# Autodesk Inventor assembly: main_pcb.brd
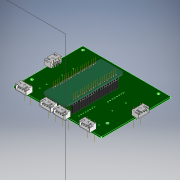
[picture p0: Inventor's stored thumbnail of the model, 180x180]
Saved by Autodesk Inventor 2022 (Build 260153000, 153)
## iProperties
Created: 2021-08-05
Part Number: main_pcb.brd
Document SubType Name: Assembly
Designer: Петров Иван
Mass: 18.6028 g
Surface Area: 275.031 cm^2
Volume: 13.5279 cm^3
Density: 1.37514 g/cm^3
Author: Петров Иван
## Documents named in this file (6)
- C:\Users\Ivan Petrov\Documents\GitHub\OmniBot\design\000.004 - Котроллер СНУ.iam
- C:\Users\Ivan Petrov\Documents\GitHub\OmniBot\design\standart_components\PBS-1.ipt
- C:\Users\Ivan Petrov\Documents\GitHub\OmniBot\design\standart_components\connectrs\JST - XH - Thru (R) - 4Pin - 2.54mm.ipt
- C:\Users\Ivan Petrov\Documents\GitHub\OmniBot\design\standart_components\CONN HEADER VERT 1POS 2.54MM.ipt
- C:\Users\Ivan Petrov\Documents\GitHub\OmniBot\design\standart_components\opencm904.ipt
- C:\Users\Ivan Petrov\Documents\GitHub\OmniBot\design\000.004.001 - Плата печатная.ipt
## Components (88 placed, 7 different names)
1. opencm904.ipt:1 — Совмещение:23, Совмещение:24, Угол:1
2. JST - XH - Thru (R) - 4Pin - 2.54mm:5 — Совмещение:37, Совмещение:38, Совмещение:39
3. JST - XH - Thru (R) - 4Pin - 2.54mm:6 — Совмещение:40, Совмещение:41, Совмещение:42
4. JST - XH - Thru (R) - 4Pin - 2.54mm:7 — Совмещение:34, Совмещение:35, Совмещение:36
5. JST - XH - Thru (R) - 4Pin - 2.54mm:10 — Совмещение:28, Совмещение:29, Совмещение:30
6. JST - XH - Thru (R) - 4Pin - 2.54mm:11 — Совмещение:31, Совмещение:32, Совмещение:33
7. 000.004.001 - Плата печатная:1 — Совмещение:25, Совмещение:26, Совмещение:27, Совмещение:28, Совмещение:29, Совмещение:30, Совмещение:31, Совмещение:32, Совмещение:33, Совмещение:34, Совмещение:35, Совмещение:36, Совмещение:37, Совмещение:38, Совмещение:39, Совмещение:40, Совмещение:41, Совмещение:42, Совмещение:43, Совмещение:44, Совмещение:45
8. JST - XH - Thru (R) - 4Pin - 2.54mm:12 — Совмещение:43, Совмещение:44, Совмещение:45
9. CONN HEADER VERT 1POS 2.54MM.ipt:1 — Совмещение:21, Совмещение:22, Заподлицо:1, Совмещение:23, Совмещение:24, Угол:1
10. PBS-1.ipt:1 — Совмещение:21, Совмещение:22, Заподлицо:1
11. CONN HEADER VERT 1POS 2.54MM:2
12. PBS-1:3
13. CONN HEADER VERT 1POS 2.54MM:3
14. PBS-1:4
15. CONN HEADER VERT 1POS 2.54MM:4
16. PBS-1:5
17. CONN HEADER VERT 1POS 2.54MM:5
18. PBS-1:6
19. CONN HEADER VERT 1POS 2.54MM:6
20. PBS-1:7
21. CONN HEADER VERT 1POS 2.54MM:7
22. PBS-1:8
23. CONN HEADER VERT 1POS 2.54MM:8
24. PBS-1:9
25. CONN HEADER VERT 1POS 2.54MM:9
26. PBS-1:10
27. CONN HEADER VERT 1POS 2.54MM:10
28. PBS-1:11
29. CONN HEADER VERT 1POS 2.54MM:11
30. PBS-1:12
31. CONN HEADER VERT 1POS 2.54MM:12
32. PBS-1:13
33. CONN HEADER VERT 1POS 2.54MM:13
34. PBS-1:14
35. CONN HEADER VERT 1POS 2.54MM:14
36. PBS-1:15
37. CONN HEADER VERT 1POS 2.54MM:15
38. PBS-1:16
39. CONN HEADER VERT 1POS 2.54MM:16
40. PBS-1:17
41. CONN HEADER VERT 1POS 2.54MM:17
42. PBS-1:18
43. CONN HEADER VERT 1POS 2.54MM:18
44. PBS-1:19
45. CONN HEADER VERT 1POS 2.54MM:19
46. PBS-1:20
47. CONN HEADER VERT 1POS 2.54MM:20
48. PBS-1:21
49. CONN HEADER VERT 1POS 2.54MM:21
50. PBS-1:22
51. CONN HEADER VERT 1POS 2.54MM:22
52. PBS-1:23
53. CONN HEADER VERT 1POS 2.54MM:23
54. PBS-1:24
55. CONN HEADER VERT 1POS 2.54MM:24
56. PBS-1:25
57. CONN HEADER VERT 1POS 2.54MM:25
58. PBS-1:26
59. CONN HEADER VERT 1POS 2.54MM:26
60. PBS-1:27
61. CONN HEADER VERT 1POS 2.54MM:27
62. PBS-1:28
63. CONN HEADER VERT 1POS 2.54MM:28
64. PBS-1:29
65. CONN HEADER VERT 1POS 2.54MM:29
66. PBS-1:30
67. CONN HEADER VERT 1POS 2.54MM:30
68. PBS-1:31
69. CONN HEADER VERT 1POS 2.54MM:31
70. PBS-1:32
71. CONN HEADER VERT 1POS 2.54MM:32
72. PBS-1:33
73. CONN HEADER VERT 1POS 2.54MM:33
74. PBS-1:34
75. CONN HEADER VERT 1POS 2.54MM:34
76. PBS-1:35
77. CONN HEADER VERT 1POS 2.54MM:35
78. PBS-1:36
79. CONN HEADER VERT 1POS 2.54MM:36
80. PBS-1:37
81. CONN HEADER VERT 1POS 2.54MM:37
82. PBS-1:38
83. CONN HEADER VERT 1POS 2.54MM:38
84. PBS-1:39
85. CONN HEADER VERT 1POS 2.54MM:39
86. PBS-1:40 — Совмещение:26, Совмещение:27
87. CONN HEADER VERT 1POS 2.54MM:40
88. PBS-1:41 — Совмещение:25
## Component patterns: (40 elements, first: CONN HEADER VERT 1POS 2.54MM.ipt:1 + PBS-1.ipt:1)
## Relationships (27: Mate 25, Flush 1, Angle 1)
- Совмещение:21 [Mate]: CONN HEADER VERT 1POS 2.54MM.ipt:1 ↔ PBS-1.ipt:1
- Совмещение:22 [Mate]: CONN HEADER VERT 1POS 2.54MM.ipt:1 ↔ PBS-1.ipt:1
- Заподлицо:1 [Flush]: CONN HEADER VERT 1POS 2.54MM.ipt:1 ↔ PBS-1.ipt:1
- Совмещение:23 [Mate]: opencm904.ipt:1 ↔ CONN HEADER VERT 1POS 2.54MM.ipt:1
- Совмещение:24 [Mate]: opencm904.ipt:1 ↔ CONN HEADER VERT 1POS 2.54MM.ipt:1
- Угол:1 [Angle] (0 deg): opencm904.ipt:1 ↔ CONN HEADER VERT 1POS 2.54MM.ipt:1
- Совмещение:25 [Mate]: 000.004.001 - Плата печатная:1 ↔ PBS-1:41
- Совмещение:26 [Mate]: 000.004.001 - Плата печатная:1 ↔ PBS-1:40
- Совмещение:27 [Mate]: 000.004.001 - Плата печатная:1 ↔ PBS-1:40
- Совмещение:28 [Mate]: JST - XH - Thru (R) - 4Pin - 2.54mm:10 ↔ 000.004.001 - Плата печатная:1
- Совмещение:29 [Mate]: JST - XH - Thru (R) - 4Pin - 2.54mm:10 ↔ 000.004.001 - Плата печатная:1
- Совмещение:30 [Mate]: JST - XH - Thru (R) - 4Pin - 2.54mm:10 ↔ 000.004.001 - Плата печатная:1
- Совмещение:31 [Mate]: JST - XH - Thru (R) - 4Pin - 2.54mm:11 ↔ 000.004.001 - Плата печатная:1
- Совмещение:32 [Mate]: JST - XH - Thru (R) - 4Pin - 2.54mm:11 ↔ 000.004.001 - Плата печатная:1
- Совмещение:33 [Mate]: JST - XH - Thru (R) - 4Pin - 2.54mm:11 ↔ 000.004.001 - Плата печатная:1
- Совмещение:34 [Mate]: JST - XH - Thru (R) - 4Pin - 2.54mm:7 ↔ 000.004.001 - Плата печатная:1
- Совмещение:35 [Mate]: JST - XH - Thru (R) - 4Pin - 2.54mm:7 ↔ 000.004.001 - Плата печатная:1
- Совмещение:36 [Mate]: JST - XH - Thru (R) - 4Pin - 2.54mm:7 ↔ 000.004.001 - Плата печатная:1
- Совмещение:37 [Mate]: JST - XH - Thru (R) - 4Pin - 2.54mm:5 ↔ 000.004.001 - Плата печатная:1
- Совмещение:38 [Mate]: JST - XH - Thru (R) - 4Pin - 2.54mm:5 ↔ 000.004.001 - Плата печатная:1
- Совмещение:39 [Mate]: JST - XH - Thru (R) - 4Pin - 2.54mm:5 ↔ 000.004.001 - Плата печатная:1
- Совмещение:40 [Mate]: JST - XH - Thru (R) - 4Pin - 2.54mm:6 ↔ 000.004.001 - Плата печатная:1
- Совмещение:41 [Mate]: JST - XH - Thru (R) - 4Pin - 2.54mm:6 ↔ 000.004.001 - Плата печатная:1
- Совмещение:42 [Mate]: JST - XH - Thru (R) - 4Pin - 2.54mm:6 ↔ 000.004.001 - Плата печатная:1
- Совмещение:43 [Mate]: 000.004.001 - Плата печатная:1 ↔ JST - XH - Thru (R) - 4Pin - 2.54mm:12
- Совмещение:44 [Mate]: 000.004.001 - Плата печатная:1 ↔ JST - XH - Thru (R) - 4Pin - 2.54mm:12
- Совмещение:45 [Mate]: 000.004.001 - Плата печатная:1 ↔ JST - XH - Thru (R) - 4Pin - 2.54mm:12
